# Autodesk Inventor assembly: manual_locker-asm
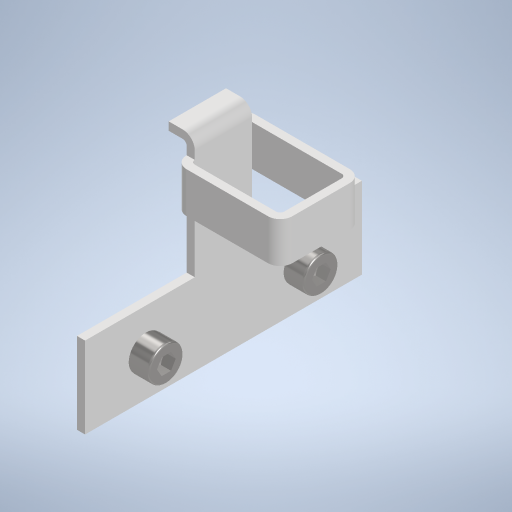
[picture p0: Inventor's stored thumbnail of the model, 512x512]
Saved by Autodesk Inventor 2024 (Build 280153000, 153)
## iProperties
Created: 2025-12-27
Part Number: manual_locker-asm
Document SubType Name: Assembly
Designer: schar
Author: schar
## Documents named in this file (4)
- C:\Users\schar\Desktop\projectBlueprint\AMSTS\hardware\manual_locker-asm.iam
- C:\Users\schar\Desktop\projectBlueprint\AMSTS\hardware\manual_locker.ipt
- C:\Users\schar\Desktop\projectBlueprint\AMSTS\hardware\tnut_m5_2020.ipt
- C:\Users\schar\Documents\Inventor\Content Center Files\R2024\en-US\ISO 4762(1)\DIN EN ISO 4762 - M5 x 8.ipt
## Components (5 placed, 3 different names)
1. manual_locker:1 — Rigid:1, Rigid:2, Mate:1, Mate:2
2. tnut_m5_2020:1 — Rigid:2, Mate:4
3. tnut_m5_2020:2 — Rigid:1, Mate:3
4. DIN EN ISO 4762 M5 x 8:1 — Mate:2, Mate:3
5. DIN EN ISO 4762 M5 x 8:2 — Mate:1, Mate:4
## Relationships (6: Mate 4, WeldJoint 2)
- Rigid:1 [WeldJoint] (0.159 mm): manual_locker:1 ↔ tnut_m5_2020:2
- Rigid:2 [WeldJoint] (0.159 mm): manual_locker:1 ↔ tnut_m5_2020:1
- Mate:1: manual_locker:1 ↔ DIN EN ISO 4762 M5 x 8:2
- Mate:2: manual_locker:1 ↔ DIN EN ISO 4762 M5 x 8:1
- Mate:3: tnut_m5_2020:2 ↔ DIN EN ISO 4762 M5 x 8:1
- Mate:4: tnut_m5_2020:1 ↔ DIN EN ISO 4762 M5 x 8:2
